# Autodesk Inventor assembly: 3t7000
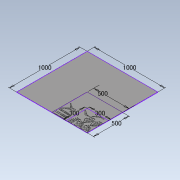
[picture p0: Inventor's stored thumbnail of the model, 180x180]
Saved by Autodesk Inventor 2020.3 (Build 243373000, 373)
## iProperties
Created: 2020-05-22
Part Number: 3t7000
Document SubType Name: Assembly
Designer: aoyama
Author: aoyama
## Documents named in this file (12)
- C:\Users\aoyam\Desktop\SRDC_local\Inventor\二年機\Geminiβ\3t7000.iam
- C:\Users\aoyam\Desktop\SRDC_local\Inventor\二年機\AL板サイズ測定板.ipt
- C:\Users\aoyam\Desktop\SRDC_local\Inventor\二年機\Geminiβ\脚\脚フレーム内側前改.ipt
- C:\Users\aoyam\Desktop\SRDC_local\Inventor\二年機\Geminiβ\脚\脚フレーム内側後改.ipt
- C:\Users\aoyam\Desktop\SRDC_local\Inventor\二年機\Geminiβ\腕\アーム揺動節test.ipt
- C:\Users\aoyam\Desktop\SRDC_local\Inventor\二年機\Geminiβ\腕\アーム中間節test.ipt
- C:\Users\aoyam\Desktop\SRDC_local\Inventor\二年機\Geminiβ\腕\アーム中間その弐.ipt
- C:\Users\aoyam\Desktop\SRDC_local\Inventor\二年機\Geminiβ\腕\中間節アーム先端締結パーツ外.ipt
- C:\Users\aoyam\Desktop\SRDC_local\Inventor\二年機\Geminiβ\腕\中間節アーム先端締結パーツ内.ipt
- C:\Users\aoyam\Desktop\SRDC_local\Inventor\二年機\Geminiβ\腕\アーム先端.ipt
- C:\Users\aoyam\Desktop\SRDC_local\Inventor\二年機\Geminiβ\汎用部品\T字金具M3long.ipt
- C:\Users\aoyam\Desktop\SRDC_local\Inventor\二年機\Geminiβ\エンドミルモデル.ipt
## Components (22 placed, 11 different names)
1. AL板サイズ測定板:1 — メイト:1, メイト:2, メイト:3, メイト:4, 角度:1, 角度:2, メイト:5, メイト:6, メイト:7, メイト:8, メイト:9, メイト:10, メイト:11, メイト:12, メイト:13, メイト:14, メイト:15, メイト:18, メイト:19, メイト:20, メイト:21, メイト:22
2. 脚フレーム内側前改:1 — メイト:2, 角度:1
3. 脚フレーム内側前改:2 — メイト:1, 角度:2
4. 脚フレーム内側後改:1 — メイト:4, メイト:5
5. 脚フレーム内側後改:2 — メイト:3, メイト:6
6. アーム揺動節test:1
7. アーム揺動節test:2
8. アーム中間節test:1 — メイト:18
9. アーム中間節test:2 — メイト:19
10. アーム中間その弐:1 — メイト:22
11. アーム中間その弐:2 — メイト:20
12. 中間節アーム先端締結パーツ外:1 — メイト:8
13. 中間節アーム先端締結パーツ内:1 — メイト:7
14. 中間節アーム先端締結パーツ外:2 — メイト:10
15. 中間節アーム先端締結パーツ内:2 — メイト:9
16. アーム先端:1 — メイト:12
17. アーム先端:2 — メイト:11
18. アーム先端:3 — フラッシュ:1, メイト:13
19. アーム先端:4 — フラッシュ:1
20. T字金具M3long:1 — メイト:14
21. T字金具M3long:2 — メイト:15
22. エンドミルモデル:1 — メイト:21
## Relationships (23: Mate 20, Angle 2, Flush 1)
- メイト:1 [Mate]: AL板サイズ測定板:1 ↔ 脚フレーム内側前改:2
- メイト:2 [Mate]: AL板サイズ測定板:1 ↔ 脚フレーム内側前改:1
- メイト:3 [Mate]: AL板サイズ測定板:1 ↔ 脚フレーム内側後改:2
- メイト:4 [Mate]: AL板サイズ測定板:1 ↔ 脚フレーム内側後改:1
- 角度:1 [Angle] (0 deg): AL板サイズ測定板:1 ↔ 脚フレーム内側前改:1
- 角度:2 [Angle] (0 deg): AL板サイズ測定板:1 ↔ 脚フレーム内側前改:2
- メイト:5 [Mate]: AL板サイズ測定板:1 ↔ 脚フレーム内側後改:1
- メイト:6 [Mate]: AL板サイズ測定板:1 ↔ 脚フレーム内側後改:2
- メイト:7 [Mate]: AL板サイズ測定板:1 ↔ 中間節アーム先端締結パーツ内:1
- メイト:8 [Mate]: AL板サイズ測定板:1 ↔ 中間節アーム先端締結パーツ外:1
- メイト:9 [Mate]: AL板サイズ測定板:1 ↔ 中間節アーム先端締結パーツ内:2
- メイト:10 [Mate]: AL板サイズ測定板:1 ↔ 中間節アーム先端締結パーツ外:2
- メイト:11 [Mate]: AL板サイズ測定板:1 ↔ アーム先端:2
- メイト:12 [Mate]: AL板サイズ測定板:1 ↔ アーム先端:1
- フラッシュ:1 [Flush]: アーム先端:3 ↔ アーム先端:4
- メイト:13 [Mate]: AL板サイズ測定板:1 ↔ アーム先端:3
- メイト:14 [Mate]: AL板サイズ測定板:1 ↔ T字金具M3long:1
- メイト:15 [Mate]: AL板サイズ測定板:1 ↔ T字金具M3long:2
- メイト:18 [Mate]: AL板サイズ測定板:1 ↔ アーム中間節test:1
- メイト:19 [Mate]: AL板サイズ測定板:1 ↔ アーム中間節test:2
- メイト:20 [Mate]: AL板サイズ測定板:1 ↔ アーム中間その弐:2
- メイト:21 [Mate]: AL板サイズ測定板:1 ↔ エンドミルモデル:1
- メイト:22 [Mate]: AL板サイズ測定板:1 ↔ アーム中間その弐:1
